# Autodesk Inventor assembly: tissue box
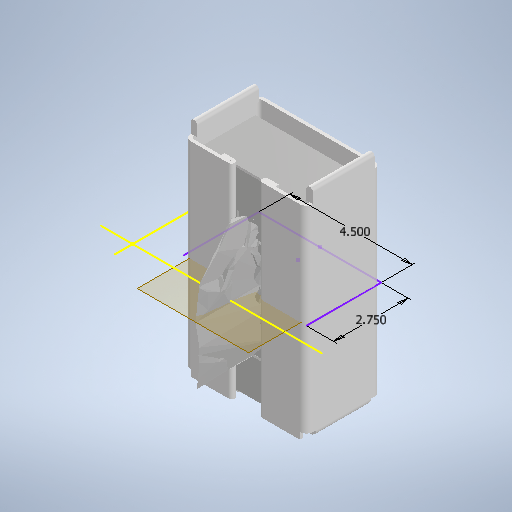
[picture p0: Inventor's stored thumbnail of the model, 512x512]
Saved by Autodesk Inventor 2025.2 (Build 292293000, 293)
## iProperties
Created: 2025-03-18
Part Number: tissue box
Document SubType Name: Assembly
Designer: bless
Author: bless
## Documents named in this file (3)
- C:\Users\bless\OneDrive - Conestoga College\Documents\Inventor\8071W25\hanging box\tissue box.iam
- C:\Users\bless\OneDrive - Conestoga College\Documents\Inventor\8071W25\stlTissueBox (1).ipt
- C:\Users\bless\OneDrive - Conestoga College\Documents\Inventor\8071W25\Hanging box.ipt
## Components (2 placed, 2 different names)
1. stlTissueBox (1):1
2. Hanging box:1 — Flush:1
## Relationships (1: Flush 1)
- Flush:1: Hanging box:1
